# Autodesk Inventor assembly: ASSEMBLY_Ballscrew
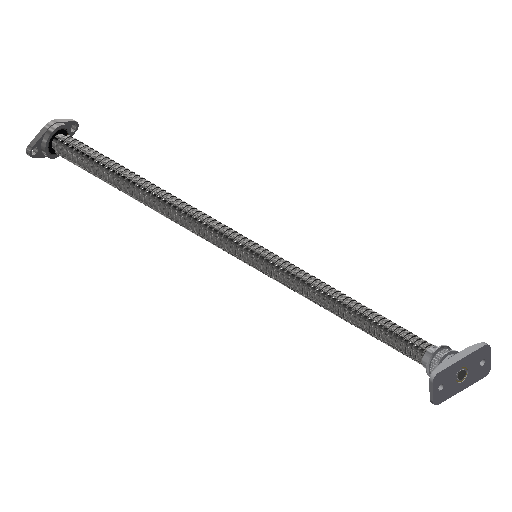
[picture p0: Inventor's stored thumbnail of the model, 512x512]
Saved by Autodesk Inventor 2026.1 (Build 301233000, 233)
## iProperties
Created: 2016-10-08
Part Number: ASSEMBLY_Ballscrew
Material: Ogólny
Document SubType Name: Assembly
Designer: Andrzej
Author: Andrzej
## Documents named in this file (7)
- C:\Users\Andrzej\OneDrive\_DRIVE_SYNCH_FILES\__ BYTECHLAB PROJECTS\MECH - FDM 3D Printer - RAPTOR-360\MCAD\1_REV1\ASSEMBLY_MAIN_REVA\ASSEMBLY_Ballscrew.iam
- C:\Users\Andrzej\OneDrive\_DRIVE_SYNCH_FILES\__ BYTECHLAB PROJECTS\MECH - FDM 3D Printer - RAPTOR-360\MCAD\1_REV1\__COTS_PARTS\COTS_GENERIC_GT2_32T_8mm_shaft_pulley.ipt
- C:\Users\Andrzej\OneDrive\_DRIVE_SYNCH_FILES\__ BYTECHLAB PROJECTS\MECH - FDM 3D Printer - RAPTOR-360\MCAD\1_REV1\__COTS_PARTS\COTS_GENERIC_SFU1605_Ball_Screw.ipt
- C:\Users\Andrzej\OneDrive\_DRIVE_SYNCH_FILES\__ BYTECHLAB PROJECTS\MECH - FDM 3D Printer - RAPTOR-360\MCAD\1_REV1\__COTS_PARTS\COTS_GENERIC_8mm_Dia_Ball_Screw_Top_Bearing_Block.ipt
- C:\Users\Andrzej\OneDrive\_DRIVE_SYNCH_FILES\__ BYTECHLAB PROJECTS\MECH - FDM 3D Printer - RAPTOR-360\MCAD\1_REV1\__COTS_PARTS\COTS_GENERIC_688HZZ_Bearing.ipt
- C:\Users\Andrzej\OneDrive\_DRIVE_SYNCH_FILES\__ BYTECHLAB PROJECTS\MECH - FDM 3D Printer - RAPTOR-360\MCAD\1_REV1\__COTS_PARTS\COTS_GENERIC_F9-20M_Bearing.ipt
- C:\Users\Andrzej\OneDrive\_DRIVE_SYNCH_FILES\__ BYTECHLAB PROJECTS\MECH - FDM 3D Printer - RAPTOR-360\MCAD\1_REV1\ASSEMBLY_MAIN_REVA\3DP_ABS_Z_Axis_Ball_Screw_Thrust_Bearing_Block.ipt
## Components (6 placed, 6 different names)
1. COTS_GENERIC_GT2_32T_8mm_shaft_pulley:1 — Zestawiający:1, Styczny:1, Zestawiający:2
2. COTS_GENERIC_SFU1605_Ball_Screw:1 — Zestawiający:1, Styczny:1, Równoległy:1, Styczny:2, Zestawiający:3, Styczny:3
3. COTS_GENERIC_8mm_Dia_Ball_Screw_Top_Bearing_Block:1 — Równoległy:1, Styczny:2, Zestawiający:6
4. COTS_GENERIC_688HZZ_Bearing:1 — Zestawiający:4, Styczny:3
5. COTS_GENERIC_F9-20M_Bearing:1 — Zestawiający:2, Zestawiający:3, Zestawiający:4, Zestawiający:5, Styczny:4
6. 3DP_ABS_Z_Axis_Ball_Screw_Thrust_Bearing_Block:1 — Zestawiający:5, Styczny:4, Zestawiający:6
## Relationships (11: Mate 6, Tangent 4, Flush 1)
- Zestawiający:1 [Mate]: COTS_GENERIC_GT2_32T_8mm_shaft_pulley:1 ↔ COTS_GENERIC_SFU1605_Ball_Screw:1
- Styczny:1 [Tangent]: COTS_GENERIC_GT2_32T_8mm_shaft_pulley:1 ↔ COTS_GENERIC_SFU1605_Ball_Screw:1
- Równoległy:1 [Flush]: COTS_GENERIC_SFU1605_Ball_Screw:1 ↔ COTS_GENERIC_8mm_Dia_Ball_Screw_Top_Bearing_Block:1
- Styczny:2 [Tangent]: COTS_GENERIC_SFU1605_Ball_Screw:1 ↔ COTS_GENERIC_8mm_Dia_Ball_Screw_Top_Bearing_Block:1
- Zestawiający:2 [Mate]: COTS_GENERIC_GT2_32T_8mm_shaft_pulley:1 ↔ COTS_GENERIC_F9-20M_Bearing:1
- Zestawiający:3 [Mate]: COTS_GENERIC_SFU1605_Ball_Screw:1 ↔ COTS_GENERIC_F9-20M_Bearing:1
- Zestawiający:4 [Mate] (0.5 mm): COTS_GENERIC_688HZZ_Bearing:1 ↔ COTS_GENERIC_F9-20M_Bearing:1
- Styczny:3 [Tangent]: COTS_GENERIC_SFU1605_Ball_Screw:1 ↔ COTS_GENERIC_688HZZ_Bearing:1
- Zestawiający:5 [Mate]: COTS_GENERIC_F9-20M_Bearing:1 ↔ 3DP_ABS_Z_Axis_Ball_Screw_Thrust_Bearing_Block:1
- Styczny:4 [Tangent]: COTS_GENERIC_F9-20M_Bearing:1 ↔ 3DP_ABS_Z_Axis_Ball_Screw_Thrust_Bearing_Block:1
- Zestawiający:6 [Mate]: COTS_GENERIC_8mm_Dia_Ball_Screw_Top_Bearing_Block:1 ↔ 3DP_ABS_Z_Axis_Ball_Screw_Thrust_Bearing_Block:1
